# Autodesk Inventor assembly: MGN12H Carriage
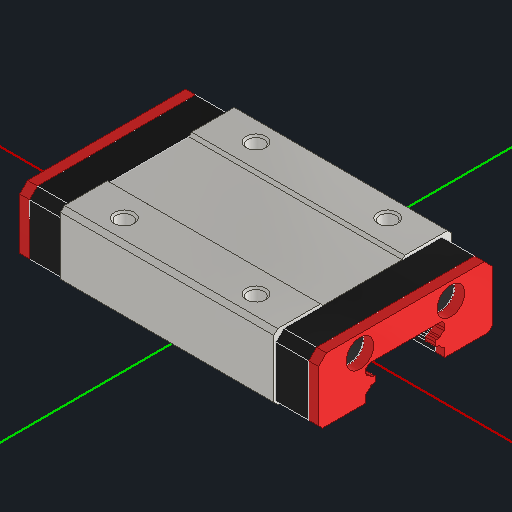
[picture p0: Inventor's stored thumbnail of the model, 512x512]
Saved by Autodesk Inventor 2022.2 (Build 262287010, 287A)
## iProperties
Created: 2022-03-15
Part Number: MGN12H Carriage
Document SubType Name: Assembly
Designer: sleib
Author: sleib
## Documents named in this file (4)
- C:\Users\sleib\Projekte\Voron-2\CAD\Inventor\MGN12H Carriage.iam
- C:\Users\sleib\Projekte\Voron-2\CAD\Inventor\MGN12H Base.ipt
- C:\Users\sleib\Projekte\Voron-2\CAD\Inventor\MGN12H End.ipt
- C:\Users\sleib\Projekte\Voron-2\CAD\Inventor\MGN12H Cap.ipt
## Components (5 placed, 3 different names)
1. MGN12H Base:1 — Fluchtend:1, Passend:1, Passend:2, Passend:3, Passend:4, Passend:5, Passend:6, Passend:9, Passend:10, Passend:13, Passend:14
2. MGN12H End:1 — Passend:6, Passend:8, Passend:13, Passend:14, Passend:15, Passend:16
3. MGN12H End:2 — Passend:5, Passend:7, Passend:9, Passend:10, Passend:11, Passend:12
4. MGN12H Cap:1 — Passend:8, Passend:15, Passend:16
5. MGN12H Cap:2 — Passend:7, Passend:11, Passend:12
## Relationships (17: Mate 16, Flush 1)
- Fluchtend:1 [Flush]: MGN12H Base:1
- Passend:1 [Mate] (10 mm): MGN12H Base:1
- Passend:2 [Mate] (10 mm): MGN12H Base:1
- Passend:3 [Mate] (-10 mm): MGN12H Base:1
- Passend:4 [Mate] (-10 mm): MGN12H Base:1
- Passend:5 [Mate]: MGN12H Base:1 ↔ MGN12H End:2
- Passend:6 [Mate]: MGN12H Base:1 ↔ MGN12H End:1
- Passend:7 [Mate]: MGN12H End:2 ↔ MGN12H Cap:2
- Passend:8 [Mate]: MGN12H End:1 ↔ MGN12H Cap:1
- Passend:9 [Mate]: MGN12H Base:1 ↔ MGN12H End:2
- Passend:10 [Mate]: MGN12H Base:1 ↔ MGN12H End:2
- Passend:11 [Mate]: MGN12H End:2 ↔ MGN12H Cap:2
- Passend:12 [Mate]: MGN12H End:2 ↔ MGN12H Cap:2
- Passend:13 [Mate]: MGN12H Base:1 ↔ MGN12H End:1
- Passend:14 [Mate]: MGN12H Base:1 ↔ MGN12H End:1
- Passend:15 [Mate]: MGN12H End:1 ↔ MGN12H Cap:1
- Passend:16 [Mate]: MGN12H End:1 ↔ MGN12H Cap:1
